# Autodesk Inventor assembly: 00 AssemblyScara
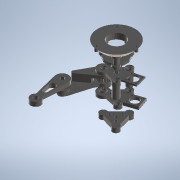
[picture p0: Inventor's stored thumbnail of the model, 180x180]
Saved by Autodesk Inventor 2020.2 (Build 242310000, 310)
## iProperties
Created: 2021-01-06
Part Number: 00 AssemblyScara
Document SubType Name: Assembly
Designer: Olivi
Author: Olivi
## Documents named in this file (18)
- C:\Users\Olivi\Universiteit Antwerpen\Plasma Robotics - General\3D parts\Parametrized+SCARA+robotic+arm.+Customizable.+1200++g+PAYLOAD+!!!\files\Total robot\Assembly\00 AssemblyScara.iam
- C:\Users\Olivi\Universiteit Antwerpen\Plasma Robotics - General\3D parts\Parametrized+SCARA+robotic+arm.+Customizable.+1200++g+PAYLOAD+!!!\files\Total robot\Assembly\01 Base.ipt
- C:\Users\Olivi\Universiteit Antwerpen\Plasma Robotics - General\3D parts\Parametrized+SCARA+robotic+arm.+Customizable.+1200++g+PAYLOAD+!!!\files\Total robot\Assembly\02 Small cil.ipt
- C:\Users\Olivi\Universiteit Antwerpen\Plasma Robotics - General\3D parts\Parametrized+SCARA+robotic+arm.+Customizable.+1200++g+PAYLOAD+!!!\files\Total robot\Assembly\03 plate .ipt
- C:\Users\Olivi\Universiteit Antwerpen\Plasma Robotics - General\3D parts\Parametrized+SCARA+robotic+arm.+Customizable.+1200++g+PAYLOAD+!!!\files\Total robot\Assembly\04 clamp x3.ipt
- C:\Users\Olivi\Universiteit Antwerpen\Plasma Robotics - General\3D parts\Parametrized+SCARA+robotic+arm.+Customizable.+1200++g+PAYLOAD+!!!\files\Total robot\Assembly\05 connectio.ipt
- C:\Users\Olivi\Universiteit Antwerpen\Plasma Robotics - General\3D parts\Parametrized+SCARA+robotic+arm.+Customizable.+1200++g+PAYLOAD+!!!\files\Total robot\Assembly\06 middle c.ipt
- C:\Users\Olivi\Universiteit Antwerpen\Plasma Robotics - General\3D parts\Parametrized+SCARA+robotic+arm.+Customizable.+1200++g+PAYLOAD+!!!\files\Total robot\Assembly\07 arm holder .ipt
- C:\Users\Olivi\Universiteit Antwerpen\Plasma Robotics - General\3D parts\Parametrized+SCARA+robotic+arm.+Customizable.+1200++g+PAYLOAD+!!!\files\Total robot\Assembly\08 arm small r.ipt
- C:\Users\Olivi\Universiteit Antwerpen\Plasma Robotics - General\3D parts\Parametrized+SCARA+robotic+arm.+Customizable.+1200++g+PAYLOAD+!!!\files\Total robot\Assembly\09 arm gear belt.ipt
- C:\Users\Olivi\Universiteit Antwerpen\Plasma Robotics - General\3D parts\Parametrized+SCARA+robotic+arm.+Customizable.+1200++g+PAYLOAD+!!!\files\Total robot\Assembly\10 arm large ri.ipt
- C:\Users\Olivi\Universiteit Antwerpen\Plasma Robotics - General\3D parts\Parametrized+SCARA+robotic+arm.+Customizable.+1200++g+PAYLOAD+!!!\files\Total robot\Assembly\11 arm holde.ipt
- C:\Users\Olivi\Universiteit Antwerpen\Plasma Robotics - General\3D parts\Parametrized+SCARA+robotic+arm.+Customizable.+1200++g+PAYLOAD+!!!\files\Total robot\Assembly\12 arm .ipt
- C:\Users\Olivi\Universiteit Antwerpen\Plasma Robotics - General\3D parts\Parametrized+SCARA+robotic+arm.+Customizable.+1200++g+PAYLOAD+!!!\files\Total robot\Assembly\13 arm end.ipt
- C:\Users\Olivi\Universiteit Antwerpen\Plasma Robotics - General\3D parts\Parametrized+SCARA+robotic+arm.+Customizable.+1200++g+PAYLOAD+!!!\files\Total robot\Assembly\14 large cil.ipt
- C:\Users\Olivi\Universiteit Antwerpen\Plasma Robotics - General\3D parts\Parametrized+SCARA+robotic+arm.+Customizable.+1200++g+PAYLOAD+!!!\files\Total robot\Assembly\15 connectio.ipt
- C:\Users\Olivi\Universiteit Antwerpen\Plasma Robotics - General\3D parts\Parametrized+SCARA+robotic+arm.+Customizable.+1200++g+PAYLOAD+!!!\files\Total robot\Assembly\16 middle c.ipt
- C:\Users\Olivi\Universiteit Antwerpen\Plasma Robotics - General\3D parts\Parametrized+SCARA+robotic+arm.+Customizable.+1200++g+PAYLOAD+!!!\files\Total robot\Assembly\17 top.ipt
## Components (22 placed, 17 different names)
1. 01 Base:1 — Mate:1, Mate:2, Mate:3, Mate:4, Mate:9, Mate:10, Mate:20, Mate:21
2. 02 Small cil:1 — Mate:1, Flush:1, Mate:5, Mate:26
3. 02 Small cil:2 — Mate:2, Flush:1, Flush:2, Mate:22, Mate:25
4. 02 Small cil:3 — Mate:3, Flush:2
5. 03 plate :1 — Mate:4, Mate:5, Mate:6, Mate:7, Mate:8
6. 04 clamp x3:1 — Mate:8, Flush:4
7. 04 clamp x3:2 — Mate:6, Flush:3, Flush:4
8. 04 clamp x3:3 — Mate:7, Flush:3
9. 05 connectio:1 — Mate:9, Mate:10, Mate:11, Mate:12, Mate:13
10. 06 middle c:1 — Mate:11, Mate:12
11. 07 arm holder :1 — Mate:13, Mate:14
12. 08 arm small r:1 — Mate:14, Mate:15
13. 09 arm gear belt:1 — Mate:15, Mate:16
14. 10 arm large ri:1 — Mate:16, Mate:17
15. 11 arm holde:1 — Mate:17, Mate:18
16. 12 arm :1 — Mate:18, Mate:19
17. 13 arm end:1 — Mate:19
18. 14 large cil:1 — Mate:21
19. 14 large cil:2 — Mate:20
20. 15 connectio:1 — Mate:22, Mate:23, Mate:24
21. 16 middle c:1 — Mate:23, Mate:24
22. 17 top:1 — Mate:25, Mate:26
## Relationships (30: Mate 26, Flush 4)
- Mate:1: 01 Base:1 ↔ 02 Small cil:1
- Mate:2: 01 Base:1 ↔ 02 Small cil:2
- Flush:1: 02 Small cil:1 ↔ 02 Small cil:2
- Mate:3: 01 Base:1 ↔ 02 Small cil:3
- Flush:2: 02 Small cil:2 ↔ 02 Small cil:3
- Mate:4: 01 Base:1 ↔ 03 plate :1
- Mate:5: 02 Small cil:1 ↔ 03 plate :1
- Mate:6: 03 plate :1 ↔ 04 clamp x3:2
- Mate:7: 03 plate :1 ↔ 04 clamp x3:3
- Mate:8: 03 plate :1 ↔ 04 clamp x3:1
- Flush:3: 04 clamp x3:2 ↔ 04 clamp x3:3
- Flush:4: 04 clamp x3:1 ↔ 04 clamp x3:2
- Mate:9: 01 Base:1 ↔ 05 connectio:1
- Mate:10: 01 Base:1 ↔ 05 connectio:1
- Mate:11: 05 connectio:1 ↔ 06 middle c:1
- Mate:12 (1.444 mm): 05 connectio:1 ↔ 06 middle c:1
- Mate:13: 05 connectio:1 ↔ 07 arm holder :1
- Mate:14: 07 arm holder :1 ↔ 08 arm small r:1
- Mate:15: 08 arm small r:1 ↔ 09 arm gear belt:1
- Mate:16: 09 arm gear belt:1 ↔ 10 arm large ri:1
- Mate:17: 10 arm large ri:1 ↔ 11 arm holde:1
- Mate:18: 11 arm holde:1 ↔ 12 arm :1
- Mate:19: 12 arm :1 ↔ 13 arm end:1
- Mate:20: 01 Base:1 ↔ 14 large cil:2
- Mate:21: 01 Base:1 ↔ 14 large cil:1
- Mate:22: 02 Small cil:2 ↔ 15 connectio:1
- Mate:23: 15 connectio:1 ↔ 16 middle c:1
- Mate:24: 15 connectio:1 ↔ 16 middle c:1
- Mate:25: 02 Small cil:2 ↔ 17 top:1
- Mate:26: 02 Small cil:1 ↔ 17 top:1
